# Autodesk Inventor assembly: Assembly_center_suspension
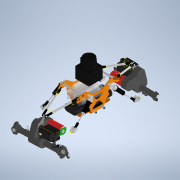
[picture p0: Inventor's stored thumbnail of the model, 180x180]
Saved by Autodesk Inventor 2020 (Build 240168000, 168)
## iProperties
Created: 2019-10-08
Part Number: Assembly_center_suspension
Document SubType Name: Assembly
Designer: maste
Author: maste
## Documents named in this file (25)
- C:\Users\maste\Documents\GitHub\autobot\robot_model\Assembly_center_suspension.iam
- C:\Users\maste\Documents\GitHub\autobot\robot_model\Assembly_center_unit.iam
- C:\Users\maste\Documents\GitHub\autobot\robot_model\RCT-H015_Tuerca_Conica.ipt
- C:\Users\maste\Documents\GitHub\autobot\robot_model\RCT-H022_washer_25_55_05.ipt
- C:\Users\maste\Documents\GitHub\autobot\robot_model\RCT-H017_lower_linkage_ball_stud.ipt
- C:\Users\maste\Documents\GitHub\autobot\robot_model\H205_lower_linkage_washer.ipt
- C:\Users\maste\Documents\GitHub\autobot\robot_model\Assembly_center_suspension\Design Accelerator\lower_linkage_ball_BC001.iam
- C:\Users\maste\Documents\GitHub\autobot\robot_model\Assembly_center_suspension\Design Accelerator\lower_linkage_ball_BC002.iam
- C:\Users\maste\Documents\GitHub\autobot\robot_model\Assembly_center_suspension\Design Accelerator\lower_linkage_ball_BC003.iam
- C:\Users\maste\Documents\GitHub\autobot\robot_model\Assembly_center_suspension\Design Accelerator\lower_linkage_ball_BC004.iam
- C:\Users\maste\Documents\GitHub\autobot\robot_model\foam_battery_base.ipt
- C:\Users\maste\Documents\GitHub\autobot\robot_model\HX-2000MHT.ipt
- C:\Users\maste\Documents\GitHub\autobot\robot_model\case_roboclaw_assembly.iam
- C:\Users\maste\Documents\GitHub\autobot\robot_model\Hokuyo Telemeter.ipt
- C:\Users\maste\Documents\GitHub\autobot\robot_model\H016 (2).ipt
- C:\Users\maste\Documents\GitHub\autobot\robot_model\Ensamblaje_eslabón.iam
- C:\Users\maste\Documents\GitHub\autobot\robot_model\Assembly_center_suspension\Design Accelerator\upper_linkage_ball_BC001.iam
- C:\Users\maste\Documents\GitHub\autobot\robot_model\RCT-H015_Bola_libertad_grande.ipt
- C:\Users\maste\Documents\GitHub\autobot\robot_model\oil_tank_Assembly.iam
- C:\Users\maste\Documents\GitHub\autobot\robot_model\piston_Assembly.iam
- C:\Users\maste\Documents\GitHub\autobot\robot_model\RCT-H017_Bola_de_libertad_menor.ipt
- C:\Users\maste\Documents\GitHub\autobot\robot_model\RCT-P002_Shock Lower Retainer 2P.ipt
- C:\Users\maste\Documents\GitHub\autobot\robot_model\front_rear_unit_assembly_fixed.iam
- C:\Users\maste\Documents\GitHub\autobot\robot_model\steering_hub_assembly.iam
- C:\Users\maste\Documents\GitHub\autobot\robot_model\steering_hub_assembly_right.iam
## Components (58 placed, 20 different names)
1. Assembly_center_unit:1 [sub-assembly] — Mate:1, Mate:2, Mate:3, Mate:4, Mate:5, Mate:6, Mate:7, Mate:8, Mate:25, Mate:26, Mate:27, Mate:28, Mate:29, Mate:30, Mate:31, Mate:32, Mate:57, Mate:58, Flush:1, Flush:2, Mate:60, Mate:61, Mate:62, Mate:63, Mate:64, Mate:65, Mate:66, Mate:67, Mate:68, Mate:69
2. RCT-H015_Tuerca_Conica:1 — Mate:1, Mate:2, Rígido:2
3. RCT-H015_Tuerca_Conica:2 — Mate:3, Mate:4, Rígido:1
4. RCT-H015_Tuerca_Conica:3 — Mate:5, Mate:6, Rígido:3
5. RCT-H015_Tuerca_Conica:4 — Mate:7, Mate:8, Rígido:4
6. RCT-H022_washer_25_55_05:1 — Mate:25, Mate:29, Mate:33, Mate:35
7. RCT-H022_washer_25_55_05:2 — Mate:26, Mate:30, Mate:34, Mate:36
8. RCT-H022_washer_25_55_05:3 — Mate:28, Mate:31, Mate:38, Mate:40
9. RCT-H022_washer_25_55_05:4 — Mate:27, Mate:32, Mate:37, Mate:39
10. RCT-H017_lower_linkage_ball_stud:1 — Mate:33, Mate:35, Mate:41, Mate:44
11. RCT-H017_lower_linkage_ball_stud:2 — Mate:34, Mate:36, Mate:42, Mate:43
12. RCT-H017_lower_linkage_ball_stud:3 — Mate:37, Mate:39, Mate:46, Mate:48
13. RCT-H017_lower_linkage_ball_stud:4 — Mate:38, Mate:40, Mate:45, Mate:47
14. H205_lower_linkage_washer:1 — Mate:41, Mate:44, Mate:51, Mate:52
15. H205_lower_linkage_washer:2 — Mate:42, Mate:43, Mate:49, Mate:50
16. H205_lower_linkage_washer:3 — Mate:45, Mate:47, Mate:55, Mate:56
17. H205_lower_linkage_washer:4 — Mate:46, Mate:48, Mate:53, Mate:54
18. Bolted Connection:5 [sub-assembly] — Mate:49, Mate:50
19. Bolted Connection:6 [sub-assembly] — Mate:51, Mate:52
20. Bolted Connection:7 [sub-assembly] — Mate:53, Mate:54
21. Bolted Connection:8 [sub-assembly] — Mate:55, Mate:56
22. foam_battery_base:1 — Mate:57, Mate:58, Flush:1, Mate:59
23. HX-2000MHT:1 — Mate:59, Flush:2
24. case_roboclaw_assembly:1 [sub-assembly]
25. Hokuyo Telemeter:1
26. H016 (2):1 — Mate:60, Mate:61, Ball:1, Angle:11
27. Ensamblaje_eslabón:1 [sub-assembly] — Ball:1, Angle:11, Ball:17, Angle:12
28. H016 (2):2 — Mate:62, Mate:63, Ball:2, Angle:2
29. Ensamblaje_eslabón:2 [sub-assembly] — Ball:2, Angle:2, Ball:18, Angle:13
30. H016 (2):3 — Mate:64, Mate:65, Ball:3, Angle:3
31. H016 (2):4 — Mate:66, Mate:67, Ball:4, Angle:4
32. Ensamblaje_eslabón:3 [sub-assembly] — Ball:3, Angle:3, Ball:16, Angle:10
33. Ensamblaje_eslabón:4 [sub-assembly] — Ball:4, Angle:4, Ball:15, Angle:9
34. Bolted Connection:9 [sub-assembly] — Mate:68, Mate:69
35. RCT-H015_Bola_libertad_grande:2 — Rígido:4, De bola:7, Ángulo:8
36. RCT-H015_Bola_libertad_grande:3 — Rígido:2, De bola:6, Ángulo:6
37. RCT-H015_Bola_libertad_grande:4 — Rígido:1, De bola:5, Ángulo:5
38. RCT-H015_Bola_libertad_grande:5 — Rígido:3, De bola:8, Ángulo:7
39. oil_tank_Assembly:1 [sub-assembly] — De bola:5, Ángulo:5, Cilíndrica:3
40. oil_tank_Assembly:2 [sub-assembly] — De bola:6, Ángulo:6, Cilíndrica:2
41. oil_tank_Assembly:3 [sub-assembly] — De bola:7, Ángulo:8, Cilíndrica:1
42. oil_tank_Assembly:4 [sub-assembly] — De bola:8, Ángulo:7, Cilíndrica:4
43. piston_Assembly:1 [sub-assembly] — Cilíndrica:2, De bola:12
44. piston_Assembly:2 [sub-assembly] — Cilíndrica:4, De bola:10
45. piston_Assembly:3 [sub-assembly] — Cilíndrica:3, De bola:11
46. piston_Assembly:4 [sub-assembly] — Cilíndrica:1, De bola:9
47. RCT-H017_Bola_de_libertad_menor:1 — De bola:10, De rotación:1
48. RCT-H017_Bola_de_libertad_menor:2 — De bola:12, De rotación:4
49. RCT-H017_Bola_de_libertad_menor:3 — De bola:11, De rotación:2
50. RCT-H017_Bola_de_libertad_menor:4 — De bola:9, De rotación:3
51. RCT-P002_Shock Lower Retainer 2P:4 — De rotación:1
52. RCT-P002_Shock Lower Retainer 2P:5 — De rotación:2
53. RCT-P002_Shock Lower Retainer 2P:6 — De rotación:3
54. RCT-P002_Shock Lower Retainer 2P:7 — De rotación:4
55. front_rear_unit_assembly_fixed:2 [sub-assembly] — Ball:15, Angle:9, Ball:16, Angle:10
56. front_rear_unit_assembly_fixed:3 [sub-assembly] — Ball:17, Angle:12, Ball:18, Angle:13, Mate:70, Mate:71, Mate:72, Mate:73
57. steering_hub_assembly:1 [sub-assembly] — Mate:70, Mate:71
58. steering_hub_assembly_right:1 [sub-assembly] — Mate:72, Mate:73
## Relationships (99: Mate 57, BallJoint 16, Angle 12, WeldJoint 4, CylindricalJoint 4, RevoluteJoint 4, Flush 2)
- Mate:1: Assembly_center_unit:1 ↔ RCT-H015_Tuerca_Conica:1
- Mate:2: Assembly_center_unit:1 ↔ RCT-H015_Tuerca_Conica:1
- Mate:3: Assembly_center_unit:1 ↔ RCT-H015_Tuerca_Conica:2
- Mate:4: Assembly_center_unit:1 ↔ RCT-H015_Tuerca_Conica:2
- Mate:5: Assembly_center_unit:1 ↔ RCT-H015_Tuerca_Conica:3
- Mate:6: Assembly_center_unit:1 ↔ RCT-H015_Tuerca_Conica:3
- Mate:7: Assembly_center_unit:1 ↔ RCT-H015_Tuerca_Conica:4
- Mate:8: Assembly_center_unit:1 ↔ RCT-H015_Tuerca_Conica:4
- Mate:25: Assembly_center_unit:1 ↔ RCT-H022_washer_25_55_05:1
- Mate:26: Assembly_center_unit:1 ↔ RCT-H022_washer_25_55_05:2
- Mate:27: Assembly_center_unit:1 ↔ RCT-H022_washer_25_55_05:4
- Mate:28: Assembly_center_unit:1 ↔ RCT-H022_washer_25_55_05:3
- Mate:29: Assembly_center_unit:1 ↔ RCT-H022_washer_25_55_05:1
- Mate:30: Assembly_center_unit:1 ↔ RCT-H022_washer_25_55_05:2
- Mate:31: Assembly_center_unit:1 ↔ RCT-H022_washer_25_55_05:3
- Mate:32: Assembly_center_unit:1 ↔ RCT-H022_washer_25_55_05:4
- Mate:33: RCT-H022_washer_25_55_05:1 ↔ RCT-H017_lower_linkage_ball_stud:1
- Mate:34: RCT-H022_washer_25_55_05:2 ↔ RCT-H017_lower_linkage_ball_stud:2
- Mate:35: RCT-H022_washer_25_55_05:1 ↔ RCT-H017_lower_linkage_ball_stud:1
- Mate:36: RCT-H022_washer_25_55_05:2 ↔ RCT-H017_lower_linkage_ball_stud:2
- Mate:37: RCT-H022_washer_25_55_05:4 ↔ RCT-H017_lower_linkage_ball_stud:3
- Mate:38: RCT-H022_washer_25_55_05:3 ↔ RCT-H017_lower_linkage_ball_stud:4
- Mate:39: RCT-H022_washer_25_55_05:4 ↔ RCT-H017_lower_linkage_ball_stud:3
- Mate:40: RCT-H022_washer_25_55_05:3 ↔ RCT-H017_lower_linkage_ball_stud:4
- Mate:41: RCT-H017_lower_linkage_ball_stud:1 ↔ H205_lower_linkage_washer:1
- Mate:42: RCT-H017_lower_linkage_ball_stud:2 ↔ H205_lower_linkage_washer:2
- Mate:43: RCT-H017_lower_linkage_ball_stud:2 ↔ H205_lower_linkage_washer:2
- Mate:44: RCT-H017_lower_linkage_ball_stud:1 ↔ H205_lower_linkage_washer:1
- Mate:45: RCT-H017_lower_linkage_ball_stud:4 ↔ H205_lower_linkage_washer:3
- Mate:46: RCT-H017_lower_linkage_ball_stud:3 ↔ H205_lower_linkage_washer:4
- Mate:47: RCT-H017_lower_linkage_ball_stud:4 ↔ H205_lower_linkage_washer:3
- Mate:48: RCT-H017_lower_linkage_ball_stud:3 ↔ H205_lower_linkage_washer:4
- Mate:49: H205_lower_linkage_washer:2 ↔ Bolted Connection:5
- Mate:50: H205_lower_linkage_washer:2 ↔ Bolted Connection:5
- Mate:51: H205_lower_linkage_washer:1 ↔ Bolted Connection:6
- Mate:52: H205_lower_linkage_washer:1 ↔ Bolted Connection:6
- Mate:53: H205_lower_linkage_washer:4 ↔ Bolted Connection:7
- Mate:54: H205_lower_linkage_washer:4 ↔ Bolted Connection:7
- Mate:55: H205_lower_linkage_washer:3 ↔ Bolted Connection:8
- Mate:56: H205_lower_linkage_washer:3 ↔ Bolted Connection:8
- Mate:57: Assembly_center_unit:1 ↔ foam_battery_base:1
- Mate:58: Assembly_center_unit:1 ↔ foam_battery_base:1
- Flush:1: Assembly_center_unit:1 ↔ foam_battery_base:1
- Mate:59: foam_battery_base:1 ↔ HX-2000MHT:1
- Flush:2 (-10 mm): Assembly_center_unit:1 ↔ HX-2000MHT:1
- Mate:60: Assembly_center_unit:1 ↔ H016 (2):1
- Mate:61: Assembly_center_unit:1 ↔ H016 (2):1
- Ball:1: H016 (2):1 ↔ Ensamblaje_eslabón:1
- Angle:11 (0 deg): H016 (2):1 ↔ Ensamblaje_eslabón:1
- Mate:62: Assembly_center_unit:1 ↔ H016 (2):2
- Mate:63: Assembly_center_unit:1 ↔ H016 (2):2
- Ball:2: H016 (2):2 ↔ Ensamblaje_eslabón:2
- Angle:2 (0 deg): H016 (2):2 ↔ Ensamblaje_eslabón:2
- Mate:64: Assembly_center_unit:1 ↔ H016 (2):3
- Mate:65: Assembly_center_unit:1 ↔ H016 (2):3
- Mate:66: Assembly_center_unit:1 ↔ H016 (2):4
- Mate:67: Assembly_center_unit:1 ↔ H016 (2):4
- Ball:3: H016 (2):3 ↔ Ensamblaje_eslabón:3
- Angle:3 (0 deg): H016 (2):3 ↔ Ensamblaje_eslabón:3
- Ball:4: H016 (2):4 ↔ Ensamblaje_eslabón:4
- Angle:4 (0 deg): H016 (2):4 ↔ Ensamblaje_eslabón:4
- Mate:68: Assembly_center_unit:1 ↔ Bolted Connection:9
- Mate:69: Assembly_center_unit:1 ↔ Bolted Connection:9
- Rígido:1 [WeldJoint]: RCT-H015_Tuerca_Conica:2 ↔ RCT-H015_Bola_libertad_grande:4
- Rígido:2 [WeldJoint]: RCT-H015_Tuerca_Conica:1 ↔ RCT-H015_Bola_libertad_grande:3
- Rígido:3 [WeldJoint]: RCT-H015_Tuerca_Conica:3 ↔ RCT-H015_Bola_libertad_grande:5
- Rígido:4 [WeldJoint]: RCT-H015_Tuerca_Conica:4 ↔ RCT-H015_Bola_libertad_grande:2
- De bola:5 [BallJoint]: RCT-H015_Bola_libertad_grande:4 ↔ oil_tank_Assembly:1
- Ángulo:5 [Angle] (0 deg): RCT-H015_Bola_libertad_grande:4 ↔ oil_tank_Assembly:1
- De bola:6 [BallJoint]: RCT-H015_Bola_libertad_grande:3 ↔ oil_tank_Assembly:2
- Ángulo:6 [Angle] (0 deg): RCT-H015_Bola_libertad_grande:3 ↔ oil_tank_Assembly:2
- De bola:7 [BallJoint]: RCT-H015_Bola_libertad_grande:2 ↔ oil_tank_Assembly:3
- De bola:8 [BallJoint]: RCT-H015_Bola_libertad_grande:5 ↔ oil_tank_Assembly:4
- Ángulo:7 [Angle] (0 deg): RCT-H015_Bola_libertad_grande:5 ↔ oil_tank_Assembly:4
- Ángulo:8 [Angle] (0 deg): RCT-H015_Bola_libertad_grande:2 ↔ oil_tank_Assembly:3
- Cilíndrica:1 [CylindricalJoint]: oil_tank_Assembly:3 ↔ piston_Assembly:4
- Cilíndrica:2 [CylindricalJoint]: oil_tank_Assembly:2 ↔ piston_Assembly:1
- Cilíndrica:3 [CylindricalJoint]: oil_tank_Assembly:1 ↔ piston_Assembly:3
- Cilíndrica:4 [CylindricalJoint]: oil_tank_Assembly:4 ↔ piston_Assembly:2
- De bola:9 [BallJoint]: piston_Assembly:4 ↔ RCT-H017_Bola_de_libertad_menor:4
- De bola:10 [BallJoint]: piston_Assembly:2 ↔ RCT-H017_Bola_de_libertad_menor:1
- De bola:11 [BallJoint]: piston_Assembly:3 ↔ RCT-H017_Bola_de_libertad_menor:3
- De bola:12 [BallJoint]: piston_Assembly:1 ↔ RCT-H017_Bola_de_libertad_menor:2
- De rotación:1 [RevoluteJoint]: RCT-H017_Bola_de_libertad_menor:1 ↔ RCT-P002_Shock Lower Retainer 2P:4
- De rotación:2 [RevoluteJoint]: RCT-H017_Bola_de_libertad_menor:3 ↔ RCT-P002_Shock Lower Retainer 2P:5
- De rotación:3 [RevoluteJoint]: RCT-H017_Bola_de_libertad_menor:4 ↔ RCT-P002_Shock Lower Retainer 2P:6
- De rotación:4 [RevoluteJoint]: RCT-H017_Bola_de_libertad_menor:2 ↔ RCT-P002_Shock Lower Retainer 2P:7
- Ball:15: Ensamblaje_eslabón:4 ↔ front_rear_unit_assembly_fixed:2
- Angle:9 (0 deg): Ensamblaje_eslabón:4 ↔ front_rear_unit_assembly_fixed:2
- Ball:16: Ensamblaje_eslabón:3 ↔ front_rear_unit_assembly_fixed:2
- Angle:10 (0 deg): Ensamblaje_eslabón:3 ↔ front_rear_unit_assembly_fixed:2
- Ball:17: Ensamblaje_eslabón:1 ↔ front_rear_unit_assembly_fixed:3
- Angle:12 (0 deg): Ensamblaje_eslabón:1 ↔ front_rear_unit_assembly_fixed:3
- Ball:18: Ensamblaje_eslabón:2 ↔ front_rear_unit_assembly_fixed:3
- Angle:13 (0 deg): Ensamblaje_eslabón:2 ↔ front_rear_unit_assembly_fixed:3
- Mate:70: front_rear_unit_assembly_fixed:3 ↔ steering_hub_assembly:1
- Mate:71 (1 mm): front_rear_unit_assembly_fixed:3 ↔ steering_hub_assembly:1
- Mate:72: front_rear_unit_assembly_fixed:3 ↔ steering_hub_assembly_right:1
- Mate:73 (1 mm): front_rear_unit_assembly_fixed:3 ↔ steering_hub_assembly_right:1
